# Autodesk Inventor assembly: robot4
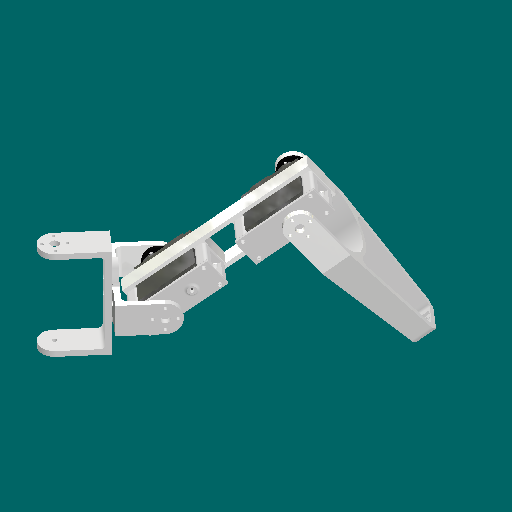
[picture p0: Inventor's stored thumbnail of the model, 512x512]
Saved by Autodesk Inventor 2026.1 (Build 301233000, 233)
## iProperties
Created: 2025-11-03
Part Number: robot4
Document SubType Name: Assembly
Designer: emanuel
Author: emanuel
## Documents named in this file (9)
- C:\Users\emanuel\UnFolder\SpiderRobo\3dmodel\leg4.iam
- C:\Users\emanuel\UnFolder\SpiderRobo\3dmodel\mg996r.ipt
- C:\Users\emanuel\UnFolder\SpiderRobo\3dmodel\servo_support_4.ipt
- C:\Users\emanuel\UnFolder\SpiderRobo\3dmodel\servo_disc.ipt
- C:\Users\emanuel\UnFolder\SpiderRobo\3dmodel\C1.ipt
- C:\Users\emanuel\UnFolder\SpiderRobo\3dmodel\smart_calf.ipt
- C:\Users\emanuel\UnFolder\SpiderRobo\3dmodel\back_servo_support.ipt
- C:\Users\emanuel\UnFolder\SpiderRobo\3dmodel\C2.ipt
- C:\Users\emanuel\UnFolder\SpiderRobo\3dmodel\femur.ipt
## Components (14 placed, 8 different names)
1. smart_calf:1 — Mate:128, Mate:129
2. servo_disc:7 — Mate:128
3. back_servo_support:3
4. C2:2 — Mate:130, Mate:131, Mate:132, Mate:133, Mate:134
5. femur:2
6. mg996r:7 — Mate:129
7. servo_disc:8
8. mg996r:8
9. back_servo_support:4
10. servo_support_4:16
11. servo_support_4:17
12. servo_support_4:18
13. servo_support_4:19
14. C1:1 — Mate:130, Mate:131, Mate:132, Mate:133, Mate:134
## Relationships (37: Mate 37)
- [Mate]: servo_disc:7 ↔ mg996r:7
- [Mate]: servo_disc:7 ↔ mg996r:7
- [Mate]: servo_disc:8 ↔ mg996r:8
- [Mate]: servo_disc:8 ↔ mg996r:8
- [Mate]: femur:2 ↔ mg996r:8
- [Mate]: femur:2 ↔ mg996r:8
- [Mate]: femur:2 ↔ mg996r:8
- [Mate]: femur:2 ↔ mg996r:7
- [Mate]: femur:2 ↔ mg996r:7
- [Mate]: femur:2 ↔ mg996r:7
- [Mate]: C2:2 ↔ servo_disc:8
- [Mate]: C2:2 ↔ mg996r:8
- [Mate]: femur:2 ↔ servo_support_4:16
- [Mate]: femur:2 ↔ servo_support_4:19
- [Mate]: femur:2 ↔ servo_support_4:17
- [Mate]: femur:2 ↔ servo_support_4:18
- [Mate]: femur:2 ↔ servo_support_4:16
- [Mate]: mg996r:7 ↔ servo_support_4:19
- [Mate]: back_servo_support:4 ↔ servo_support_4:16
- [Mate]: back_servo_support:4 ↔ servo_support_4:16
- [Mate]: back_servo_support:4 ↔ servo_support_4:16
- [Mate]: back_servo_support:4 ↔ servo_support_4:19
- [Mate]: femur:2 ↔ servo_support_4:16
- [Mate]: femur:2 ↔ servo_support_4:18
- [Mate]: femur:2 ↔ servo_support_4:18
- [Mate]: mg996r:8 ↔ servo_support_4:17
- [Mate]: back_servo_support:3 ↔ servo_support_4:18
- [Mate]: back_servo_support:3 ↔ servo_support_4:18
- [Mate]: back_servo_support:3 ↔ servo_support_4:18
- [Mate]: back_servo_support:3 ↔ servo_support_4:17
- Mate:128: smart_calf:1 ↔ servo_disc:7
- Mate:129: smart_calf:1 ↔ mg996r:7
- Mate:130: C2:2 ↔ C1:1
- Mate:131: C2:2 ↔ C1:1
- Mate:132: C2:2 ↔ C1:1
- Mate:133: C2:2 ↔ C1:1
- Mate:134: C2:2 ↔ C1:1
## Named parameters: d125_d101 = 0 mm, d126_d102 = 0 mm, d127_d103 = 0 mm, d128_d104 = 0 mm, d129_d105 = 0 mm, d130_d106 = 0 mm, d131_d107 = 0 mm, d132_d108 = 0 mm, d133_d109 = 0 mm, d134_d110 = 0 mm, d135_d111 = 0 mm, d136_d112 = 0 mm, d137_d113 = 0 mm, d138_d114 = 0 mm, d139_d115 = 0 mm, d140_d116 = 0 mm, d141_d117 = 0 mm, d142_d118 = 0 mm, d143_d119 = 0 mm, d144_d120 = 0 mm, d145_d121 = 0 mm, d146_d122 = 0 mm, d147_d123 = 0 mm, d148_d124 = 0 mm, d149_d95 = 0 mm, d150_d96 = 0 mm, d151_d97_d95 = 0 mm, d152_d98_d96 = 0 mm, d153_d99 = 0 mm, d154_d100 = 0 mm
